# Autodesk Inventor assembly: 17-0028-0020
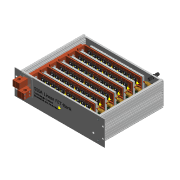
[picture p0: Inventor's stored thumbnail of the model, 180x180]
Saved by Autodesk Inventor 2016 SP2 (Build 200236200, 236)
## iProperties
Created: 2017-11-01
Part Number: 17-0028-0020
Document SubType Name: Assembly
Designer: Daan Giesen
Mass: 18489.3 g
Surface Area: 29986.8 cm^2
Volume: 4293.15 cm^3
Density: 4.30669 g/cm^3
Project: Digital PID Loop
Cost Center: 17-0028
User Status: Work in Progress
Authority: Reichsöllner, Lukas
Description: FET bank array
RuleStatus: InUse
Category: -
Company: Universiteit van Amsterdam
BeforeDocSave0: Show Form
Author: Daan Giesen
Title: Digital PID Loop
Revision Number: A
## Documents named in this file (11)
- D:\VaultLocalWorkingFolder\UvA_MT\Projects\2017\17-0028 Digital PID Loop\10_Assemblies\17-0028-0020.iam
- D:\VaultLocalWorkingFolder\UvA_MT\Projects\2017\17-0028 Digital PID Loop\10_Assemblies\17-0028-0019.iam
- D:\VaultLocalWorkingFolder\UvA_MT\Projects\2017\17-0028 Digital PID Loop\20_3D-Models\17-0028-0079.iam
- D:\VaultLocalWorkingFolder\UvA_MT\Projects\2017\17-0028 Digital PID Loop\20_3D-Models\17-0028-0061.iam
- D:\VaultLocalWorkingFolder\UvA_MT\Projects\2017\17-0028 Digital PID Loop\10_Assemblies\17-0028-0099.iam
- D:\VaultLocalWorkingFolder\UvA_MT\Projects\2017\17-0028 Digital PID Loop\10_Assemblies\17-0028-0020\Design Accelerator\17-0028-0106.iam
- D:\VaultLocalWorkingFolder\UvA_MT\Projects\2017\17-0028 Digital PID Loop\10_Assemblies\17-0028-0020\Design Accelerator\101530.iam
- D:\VaultLocalWorkingFolder\UvA_MT\Projects\2017\17-0028 Digital PID Loop\10_Assemblies\17-0028-0020\Design Accelerator\17-0028-0108.iam
- D:\VaultLocalWorkingFolder\UvA_MT\Projects\2017\17-0028 Digital PID Loop\20_3D-Models\17-0028-0112.ipt
- D:\VaultLocalWorkingFolder\UvA_MT\UVA_library\Serto\SO 31521-6 168_1500_060.ipt
- D:\VaultLocalWorkingFolder\UvA_MT\Projects\2017\17-0028 Digital PID Loop\20_3D-Models\CA_3_GS.ipt
## Components (27 placed, 8 different names)
1. 17-0028-0079:1 [sub-assembly] — Mate:6, Mate:7, Mate:10, Mate:11, Mate:12, Mate:29, Mate:30
2. 17-0028-0061:1 [sub-assembly] — Mate:10, Mate:11, Mate:12, Mate:31, Mate:32, Mate:33, Mate:34, Mate:35, Mate:36, Mate:37, Mate:38, Mate:39
3. 17-0028-0099:1 [sub-assembly] — Flush:1, Mate:21, Flush:3, Mate:27
4. 17-0028-0099:2 [sub-assembly] — Flush:2, Mate:22, Flush:4, Mate:25
5. Bolted Connection:18 [sub-assembly] — Mate:29, Mate:30
6. 17-0028-0112:1 — Mate:31, Mate:32, Mate:33
7. SO 31521-6 168_1500_060:1 — Mate:35, Mate:37
8. SO 31521-6 168_1500_060:2 — Mate:34, Mate:36
9. CA_3_GS:1 — Mate:38, Mate:39
10. 17-0028-0019:1 [sub-assembly] — Mate:6, Mate:7, Mate:21, Flush:3, Mate:22, Flush:4
11. 17-0028-0019:2 [sub-assembly]
12. 17-0028-0019:3 [sub-assembly]
13. 17-0028-0019:4 [sub-assembly]
14. 17-0028-0019:5 [sub-assembly]
15. 17-0028-0019:6 [sub-assembly] — Flush:1, Flush:2, Mate:26, Mate:28
16. Bolted Connection:1 [sub-assembly] — Mate:27, Mate:28
17. Bolted Connection:7 [sub-assembly] — Mate:25, Mate:26
18. Bolted Connection:8 [sub-assembly]
19. Bolted Connection:9 [sub-assembly]
20. Bolted Connection:10 [sub-assembly]
21. Bolted Connection:11 [sub-assembly]
22. Bolted Connection:12 [sub-assembly]
23. Bolted Connection:13 [sub-assembly]
24. Bolted Connection:14 [sub-assembly]
25. Bolted Connection:15 [sub-assembly]
26. Bolted Connection:16 [sub-assembly]
27. Bolted Connection:17 [sub-assembly]
## Component patterns: (6 elements, first: 17-0028-0019:1), (6 elements, first: Bolted Connection:1 + Bolted Connection:7)
## Relationships (26: Mate 22, Flush 4)
- Mate:6 (60 mm): 17-0028-0079:1 ↔ 17-0028-0019:1
- Mate:7: 17-0028-0079:1 ↔ 17-0028-0019:1
- Mate:10 (1 mm): 17-0028-0079:1 ↔ 17-0028-0061:1
- Mate:11: 17-0028-0079:1 ↔ 17-0028-0061:1
- Mate:12: 17-0028-0079:1 ↔ 17-0028-0061:1
- Flush:1: 17-0028-0099:1 ↔ 17-0028-0019:6
- Flush:2: 17-0028-0099:2 ↔ 17-0028-0019:6
- Mate:21: 17-0028-0099:1 ↔ 17-0028-0019:1
- Flush:3: 17-0028-0099:1 ↔ 17-0028-0019:1
- Mate:22: 17-0028-0099:2 ↔ 17-0028-0019:1
- Flush:4: 17-0028-0099:2 ↔ 17-0028-0019:1
- Mate:25: 17-0028-0099:2 ↔ Bolted Connection:7
- Mate:26: 17-0028-0019:6 ↔ Bolted Connection:7
- Mate:27: 17-0028-0099:1 ↔ Bolted Connection:1
- Mate:28: 17-0028-0019:6 ↔ Bolted Connection:1
- Mate:29: 17-0028-0079:1 ↔ Bolted Connection:18
- Mate:30: 17-0028-0079:1 ↔ Bolted Connection:18
- Mate:31 (-10 mm): 17-0028-0061:1 ↔ 17-0028-0112:1
- Mate:32: 17-0028-0061:1 ↔ 17-0028-0112:1
- Mate:33 (-10 mm): 17-0028-0061:1 ↔ 17-0028-0112:1
- Mate:34: 17-0028-0061:1 ↔ SO 31521-6 168_1500_060:2
- Mate:35: 17-0028-0061:1 ↔ SO 31521-6 168_1500_060:1
- Mate:36: 17-0028-0061:1 ↔ SO 31521-6 168_1500_060:2
- Mate:37: 17-0028-0061:1 ↔ SO 31521-6 168_1500_060:1
- Mate:38: 17-0028-0061:1 ↔ CA_3_GS:1
- Mate:39: 17-0028-0061:1 ↔ CA_3_GS:1
